# Autodesk Inventor assembly: AK-C-C39-vertival
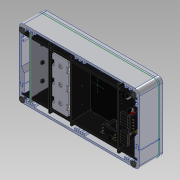
[picture p0: Inventor's stored thumbnail of the model, 180x180]
Saved by Autodesk Inventor 2016 (Build 200138000, 138)
## iProperties
Created: 2016-04-02
Part Number: AK-C-C39-vertival
Document SubType Name: Assembly
Designer: admin
Author: admin
## Documents named in this file (21)
- E:\Alex\DI-Lambda\parts\v1\AK-C-C39\AK-C-C39-DI-Lambda-v1.iam
- E:\Alex\DI-Lambda\parts\Common\SZOMK-AK-C-C39.ipt
- E:\Alex\DI-Lambda\parts\v1\AK-C-C39\AK-C-C39-Top.ipt
- E:\Alex\DI-Lambda\parts\v1\AK-C-C39\AK-C-C39-Main-Board.ipt
- E:\Alex\DI-Lambda\parts\v1\AK-C-C39\AK-C-C39-Separator.ipt
- E:\Alex\DI-Lambda\parts\v1\AK-C-C39\AK-C-C39-Pinhole-Board.ipt
- E:\Alex\DI-Lambda\parts\v1\AK-C-C39\AK-C-C39-LED-Board-Assembly.iam
- E:\Alex\DI-Lambda\parts\v1\AK-C-C39\AK-C-C39-Sensor-Board.ipt
- E:\Alex\DI-Lambda\parts\v1\AK-C-C39\AK-C-C39-Bottom.ipt
- E:\Alex\DI-Lambda\parts\Common\Cuvette.ipt
- E:\Alex\DI-Lambda\parts\Common\Paper-holder.iam
- E:\Alex\DI-Lambda\parts\v1\AK-C-C39\LCD.ipt
- E:\Alex\DI-Lambda\parts\Common\Button.ipt
- C:\Users\admin\Documents\Inventor\Content Center Files\R2016\en-US\SS-ISO 7046  Z\ISO 7046-1 - M3 x 8Z.ipt
- E:\Alex\DI-Lambda\parts\v1\AK-C-C39\AK-C-C39-Holder-IM.ipt
- E:\Alex\DI-Lambda\parts\v1\AK-C-C39\AK-C-C39-LED-Board-Assembly2.iam
- E:\Alex\DI-Lambda\parts\Common\fciconnect-91601-304.ipt
- E:\Alex\DI-Lambda\parts\v1\AK-C-C39\AK-C-C39-USB-Board-Assembly.iam
- E:\Alex\DI-Lambda\parts\v1\AK-C-C39\AK-C-C39-LED-Module.iam
- C:\Users\admin\Documents\Inventor\Content Center Files\R2016\en-US\ISO 1580\ISO 1580 - M2 x 5.ipt
- C:\Users\admin\Documents\Inventor\Content Center Files\R2016\en-US\ISO 8738(2)\ISO 8738 - 3(2).ipt
## Components (37 placed, 20 different names)
1. SZOMK-AK-C-C39:1 — Mate:1, Mate:2, Mate:3, Mate:117, Mate:118, Mate:119
2. AK-C-C39-Top:1 — Mate:1, Mate:2, Mate:3, Mate:4, Mate:68, Mate:69, Mate:70, Mate:71, Flush:1, Flush:2, Flush:3, Flush:4, Mate:86, Mate:87, Mate:98, Mate:99, Mate:132, Mate:133
3. AK-C-C39-Main-Board:1 — Mate:4, Mate:25, Mate:29, Mate:30, Mate:32, Mate:33, Mate:35, Mate:47, Mate:50, Mate:51, Mate:52, Mate:53, Mate:54, Mate:55, Mate:84, Mate:85, Mate:86, Mate:87, Mate:88, Mate:89, Mate:90, Mate:91, Mate:92, Mate:93, Mate:94, Mate:96, Mate:97, Mate:100, Mate:101, Mate:102, Mate:103, Mate:104, Angle:1, Angle:2, Mate:109, Mate:116, Mate:126, Mate:127, Mate:128, Mate:129
4. AK-C-C39-Separator:1 — Mate:25, Mate:85, Mate:94
5. AK-C-C39-Separator:2 — Mate:35, Mate:84
6. AK-C-C39-LED-Board-Assembly:1 [sub-assembly] — Mate:32, Mate:33, Mate:96
7. AK-C-C39-Sensor-Board:1 — Mate:29, Mate:30, Mate:100
8. AK-C-C39-Bottom:1 — Mate:117, Mate:118, Mate:119, Mate:122, Mate:123, Mate:124, Mate:125, Flush:7, Flush:8, Flush:9, Flush:10
9. Cuvette:1
10. Paper-holder:1 [sub-assembly]
11. LCD:1 — Mate:47
12. Button:1 — Mate:50
13. Button:2 — Mate:51
14. Button:3 — Mate:52
15. Button:4 — Mate:53
16. Button:5 — Mate:54
17. Button:6 — Mate:55
18. SS ISO 7046 Z M3 x 8:1 — Mate:68, Flush:1
19. SS ISO 7046 Z M3 x 8:2 — Mate:69, Flush:2
20. SS ISO 7046 Z M3 x 8:3 — Mate:70, Flush:3
21. SS ISO 7046 Z M3 x 8:4 — Mate:71, Flush:4
22. SS ISO 7046 Z M3 x 8:5 — Mate:122, Flush:8
23. SS ISO 7046 Z M3 x 8:6 — Mate:124, Flush:10
24. SS ISO 7046 Z M3 x 8:7 — Mate:123, Flush:7
25. SS ISO 7046 Z M3 x 8:8 — Mate:125, Flush:9
26. AK-C-C39-Pinhole-Board:1 — Mate:88, Mate:90, Mate:91
27. AK-C-C39-Pinhole-Board:2 — Mate:89, Mate:92, Mate:93
28. AK-C-C39-Holder-IM:1 — Mate:97, Mate:98, Mate:99
29. AK-C-C39-LED-Board-Assembly2:1 [sub-assembly] — Mate:101, Mate:102, Mate:103, Mate:120, Tangent:1, Angle:3, Mate:121
30. fciconnect-91601-304:1 — Flush:5, Mate:104, Flush:6, Angle:1, Mate:105, Mate:108
31. fciconnect-91601-304:2 — Flush:5, Flush:6, Mate:106, Mate:107
32. AK-C-C39-USB-Board-Assembly:1 [sub-assembly] — Angle:2, Mate:105, Mate:106, Mate:107, Mate:108, Mate:109, Mate:110, Mate:111, Mate:112, Mate:113, Mate:114, Mate:115
33. AK-C-C39-LED-Module:1 [sub-assembly] — Mate:120, Tangent:1, Angle:3, Mate:121
34. ISO 1580 M2 x 5:1 — Mate:130, Mate:132
35. ISO 1580 M2 x 5:2 — Mate:131, Mate:133
36. ISO 8738 3:1 — Mate:127, Mate:129, Mate:131
37. ISO 8738 3:2 — Mate:126, Mate:128, Mate:130
## Relationships (84: Mate 70, Flush 10, Angle 3, Tangent 1)
- Mate:1: SZOMK-AK-C-C39:1 ↔ AK-C-C39-Top:1
- Mate:2: SZOMK-AK-C-C39:1 ↔ AK-C-C39-Top:1
- Mate:3: SZOMK-AK-C-C39:1 ↔ AK-C-C39-Top:1
- Mate:4: AK-C-C39-Top:1 ↔ AK-C-C39-Main-Board:1
- Mate:25: AK-C-C39-Main-Board:1 ↔ AK-C-C39-Separator:1
- Mate:29: AK-C-C39-Main-Board:1 ↔ AK-C-C39-Sensor-Board:1
- Mate:30: AK-C-C39-Main-Board:1 ↔ AK-C-C39-Sensor-Board:1
- Mate:32: AK-C-C39-Main-Board:1 ↔ AK-C-C39-LED-Board-Assembly:1
- Mate:33: AK-C-C39-Main-Board:1 ↔ AK-C-C39-LED-Board-Assembly:1
- Mate:35: AK-C-C39-Main-Board:1 ↔ AK-C-C39-Separator:2
- Mate:47: AK-C-C39-Main-Board:1 ↔ LCD:1
- Mate:50: AK-C-C39-Main-Board:1 ↔ Button:1
- Mate:51: AK-C-C39-Main-Board:1 ↔ Button:2
- Mate:52: AK-C-C39-Main-Board:1 ↔ Button:3
- Mate:53: AK-C-C39-Main-Board:1 ↔ Button:4
- Mate:54: AK-C-C39-Main-Board:1 ↔ Button:5
- Mate:55: AK-C-C39-Main-Board:1 ↔ Button:6
- Mate:68: AK-C-C39-Top:1 ↔ SS ISO 7046 Z M3 x 8:1
- Mate:69: AK-C-C39-Top:1 ↔ SS ISO 7046 Z M3 x 8:2
- Mate:70: AK-C-C39-Top:1 ↔ SS ISO 7046 Z M3 x 8:3
- Mate:71: AK-C-C39-Top:1 ↔ SS ISO 7046 Z M3 x 8:4
- Flush:1: AK-C-C39-Top:1 ↔ SS ISO 7046 Z M3 x 8:1
- Flush:2: AK-C-C39-Top:1 ↔ SS ISO 7046 Z M3 x 8:2
- Flush:3: AK-C-C39-Top:1 ↔ SS ISO 7046 Z M3 x 8:3
- Flush:4: AK-C-C39-Top:1 ↔ SS ISO 7046 Z M3 x 8:4
- Mate:84: AK-C-C39-Main-Board:1 ↔ AK-C-C39-Separator:2
- Mate:85: AK-C-C39-Main-Board:1 ↔ AK-C-C39-Separator:1
- Mate:86: AK-C-C39-Top:1 ↔ AK-C-C39-Main-Board:1
- Mate:87: AK-C-C39-Top:1 ↔ AK-C-C39-Main-Board:1
- Mate:88: AK-C-C39-Main-Board:1 ↔ AK-C-C39-Pinhole-Board:1
- Mate:89: AK-C-C39-Main-Board:1 ↔ AK-C-C39-Pinhole-Board:2
- Mate:90: AK-C-C39-Main-Board:1 ↔ AK-C-C39-Pinhole-Board:1
- Mate:91: AK-C-C39-Main-Board:1 ↔ AK-C-C39-Pinhole-Board:1
- Mate:92: AK-C-C39-Main-Board:1 ↔ AK-C-C39-Pinhole-Board:2
- Mate:93: AK-C-C39-Main-Board:1 ↔ AK-C-C39-Pinhole-Board:2
- Mate:94: AK-C-C39-Main-Board:1 ↔ AK-C-C39-Separator:1
- Mate:96: AK-C-C39-Main-Board:1 ↔ AK-C-C39-LED-Board-Assembly:1
- Mate:97: AK-C-C39-Main-Board:1 ↔ AK-C-C39-Holder-IM:1
- Mate:98: AK-C-C39-Top:1 ↔ AK-C-C39-Holder-IM:1
- Mate:99: AK-C-C39-Top:1 ↔ AK-C-C39-Holder-IM:1
- Mate:100: AK-C-C39-Main-Board:1 ↔ AK-C-C39-Sensor-Board:1
- Mate:101: AK-C-C39-Main-Board:1 ↔ AK-C-C39-LED-Board-Assembly2:1
- Mate:102: AK-C-C39-Main-Board:1 ↔ AK-C-C39-LED-Board-Assembly2:1
- Mate:103: AK-C-C39-Main-Board:1 ↔ AK-C-C39-LED-Board-Assembly2:1
- Flush:5: fciconnect-91601-304:1 ↔ fciconnect-91601-304:2
- Mate:104: AK-C-C39-Main-Board:1 ↔ fciconnect-91601-304:1
- Flush:6: fciconnect-91601-304:1 ↔ fciconnect-91601-304:2
- Angle:1 (0 deg): AK-C-C39-Main-Board:1 ↔ fciconnect-91601-304:1
- Angle:2 (0 deg): AK-C-C39-Main-Board:1 ↔ AK-C-C39-USB-Board-Assembly:1
- Mate:105: fciconnect-91601-304:1 ↔ AK-C-C39-USB-Board-Assembly:1
- Mate:106 (0.25 mm): fciconnect-91601-304:2 ↔ AK-C-C39-USB-Board-Assembly:1
- Mate:107 (0.25 mm): fciconnect-91601-304:2 ↔ AK-C-C39-USB-Board-Assembly:1
- Mate:108 (0.25 mm): fciconnect-91601-304:1 ↔ AK-C-C39-USB-Board-Assembly:1
- Mate:109 (0.5 mm): AK-C-C39-Main-Board:1 ↔ AK-C-C39-USB-Board-Assembly:1
- Mate:110: AK-C-C39-USB-Board-Assembly:1
- Mate:111: AK-C-C39-USB-Board-Assembly:1
- Mate:112: AK-C-C39-USB-Board-Assembly:1
- Mate:113: AK-C-C39-USB-Board-Assembly:1
- Mate:114: AK-C-C39-USB-Board-Assembly:1
- Mate:115: AK-C-C39-USB-Board-Assembly:1
- Mate:116: AK-C-C39-Main-Board:1
- Mate:117: SZOMK-AK-C-C39:1 ↔ AK-C-C39-Bottom:1
- Mate:118: SZOMK-AK-C-C39:1 ↔ AK-C-C39-Bottom:1
- Mate:119: SZOMK-AK-C-C39:1 ↔ AK-C-C39-Bottom:1
- Mate:120: AK-C-C39-LED-Board-Assembly2:1 ↔ AK-C-C39-LED-Module:1
- Tangent:1: AK-C-C39-LED-Board-Assembly2:1 ↔ AK-C-C39-LED-Module:1
- Angle:3 (0 deg): AK-C-C39-LED-Board-Assembly2:1 ↔ AK-C-C39-LED-Module:1
- Mate:121: AK-C-C39-LED-Board-Assembly2:1 ↔ AK-C-C39-LED-Module:1
- Mate:122: AK-C-C39-Bottom:1 ↔ SS ISO 7046 Z M3 x 8:5
- Mate:123: AK-C-C39-Bottom:1 ↔ SS ISO 7046 Z M3 x 8:7
- Mate:124: AK-C-C39-Bottom:1 ↔ SS ISO 7046 Z M3 x 8:6
- Mate:125: AK-C-C39-Bottom:1 ↔ SS ISO 7046 Z M3 x 8:8
- Flush:7: AK-C-C39-Bottom:1 ↔ SS ISO 7046 Z M3 x 8:7
- Flush:8: AK-C-C39-Bottom:1 ↔ SS ISO 7046 Z M3 x 8:5
- Flush:9: AK-C-C39-Bottom:1 ↔ SS ISO 7046 Z M3 x 8:8
- Flush:10: AK-C-C39-Bottom:1 ↔ SS ISO 7046 Z M3 x 8:6
- Mate:126: AK-C-C39-Main-Board:1 ↔ ISO 8738 3:2
- Mate:127: AK-C-C39-Main-Board:1 ↔ ISO 8738 3:1
- Mate:128: AK-C-C39-Main-Board:1 ↔ ISO 8738 3:2
- Mate:129: AK-C-C39-Main-Board:1 ↔ ISO 8738 3:1
- Mate:130: ISO 1580 M2 x 5:1 ↔ ISO 8738 3:2
- Mate:131: ISO 1580 M2 x 5:2 ↔ ISO 8738 3:1
- Mate:132: AK-C-C39-Top:1 ↔ ISO 1580 M2 x 5:1
- Mate:133: AK-C-C39-Top:1 ↔ ISO 1580 M2 x 5:2
